# Autodesk Inventor assembly: ASY DMF filter package v2.1
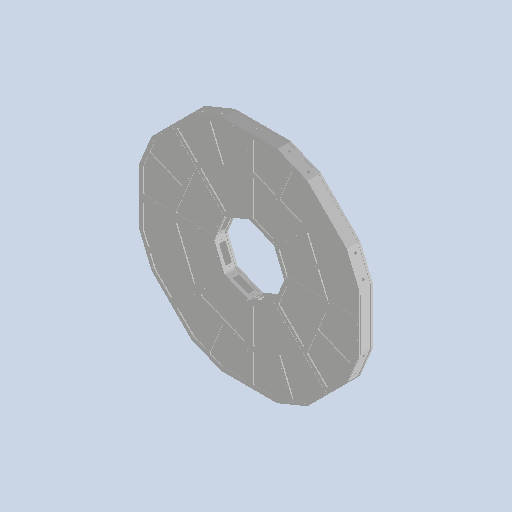
[picture p0: Inventor's stored thumbnail of the model, 512x512]
Saved by Autodesk Inventor 2025 (Build 290162010, 162A)
## iProperties
Created: 2024-05-16
Part Number: ASY DMF filter package v2.1
Document SubType Name: Assembly
Designer: admin
Author: admin
## Documents named in this file (2)
- C:\Users\pokla\Documents\Inventor\ДФО\ДМФ\DMF-Disk-Micro-Filter\Барабан v2.1\ASY DMF filter package v2.1.iam
- C:\Users\pokla\Documents\Inventor\ДФО\ДМФ\DMF-Disk-Micro-Filter\Барабан v2.1\ASY DMF 01 50 tape v2.1.iam
## Components (8 placed, 1 different names)
1. ASY DMF 01 50 tape v2.1.iam:1 [sub-assembly] — Mate:1, Flush:1
2. ASY DMF 01 50 tape v2.1.iam:2 [sub-assembly]
3. ASY DMF 01 50 tape v2.1.iam:3 [sub-assembly] — Flush:2
4. ASY DMF 01 50 tape v2.1.iam:4 [sub-assembly]
5. ASY DMF 01 50 tape v2.1.iam:5 [sub-assembly]
6. ASY DMF 01 50 tape v2.1.iam:6 [sub-assembly]
7. ASY DMF 01 50 tape v2.1.iam:7 [sub-assembly]
8. ASY DMF 01 50 tape v2.1.iam:8 [sub-assembly]
## Relationships (10: WeldJoint 7, Flush 2, Mate 1)
- [WeldJoint]: ASY DMF 01 50 tape v2.1.iam:1 ↔ ASY DMF 01 50 tape v2.1.iam:2
- [WeldJoint]: ASY DMF 01 50 tape v2.1.iam:2 ↔ ASY DMF 01 50 tape v2.1.iam:3
- [WeldJoint]: ASY DMF 01 50 tape v2.1.iam:3 ↔ ASY DMF 01 50 tape v2.1.iam:4
- [WeldJoint]: ASY DMF 01 50 tape v2.1.iam:4 ↔ ASY DMF 01 50 tape v2.1.iam:5
- [WeldJoint]: ASY DMF 01 50 tape v2.1.iam:5 ↔ ASY DMF 01 50 tape v2.1.iam:6
- [WeldJoint]: ASY DMF 01 50 tape v2.1.iam:6 ↔ ASY DMF 01 50 tape v2.1.iam:7
- [WeldJoint]: ASY DMF 01 50 tape v2.1.iam:7 ↔ ASY DMF 01 50 tape v2.1.iam:8
- Mate:1: ASY DMF 01 50 tape v2.1.iam:1
- Flush:1: ASY DMF 01 50 tape v2.1.iam:1
- Flush:2: ASY DMF 01 50 tape v2.1.iam:3
